# Autodesk Inventor assembly: Butterfly Drive Module
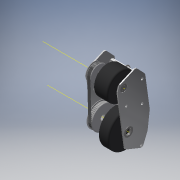
[picture p0: Inventor's stored thumbnail of the model, 180x180]
Saved by Autodesk Inventor 2019.4 (Build 234330000, 330)
## iProperties
Created: 2019-11-02
Part Number: Butterfly Drive Module
Document SubType Name: Assembly
Designer: admin
Author: admin
## Documents named in this file (12)
- C:\Users\admin\Desktop\FRC 2020 Engineering\GitHub\7738-CAD-prep\Butterfly Drive Mk2\Butterfly Module\Butterfly Drive Module.iam
- C:\Users\admin\Desktop\FRC 2020 Engineering\GitHub\7738-CAD-prep\Butterfly Drive Mk2\Butterfly Module\100mm Mecanum StandIn.ipt
- C:\Users\admin\Desktop\FRC 2020 Engineering\GitHub\7738-CAD-prep\Butterfly Drive Mk2\Butterfly Module\100mm Traction Wheel StandIn.ipt
- C:\Users\admin\Desktop\FRC 2020 Engineering\GitHub\7738-CAD-prep\Butterfly Drive Mk2\Butterfly Module\Connector.ipt
- C:\Users\admin\Desktop\FRC 2020 Engineering\GitHub\7738-CAD-prep\Butterfly Drive Mk2\Butterfly Module\F6802.ipt
- C:\Users\admin\Desktop\FRC 2020 Engineering\GitHub\7738-CAD-prep\Butterfly Drive Mk2\Butterfly Module\M6GBTeye.ipt
- C:\Users\admin\Desktop\FRC 2020 Engineering\GitHub\7738-CAD-prep\Butterfly Drive Mk2\Butterfly Module\Module Plate 1.ipt
- C:\Users\admin\Desktop\FRC 2020 Engineering\GitHub\7738-CAD-prep\Butterfly Drive Mk2\Butterfly Module\Butterfly Drive Module\Design Accelerator\Synchronous Belts Transmission1.iam
- C:\Users\admin\Desktop\FRC 2020 Engineering\GitHub\7738-CAD-prep\Butterfly Drive Mk2\Butterfly Module\Pneumatics Connector.ipt
- C:\Users\admin\Desktop\FRC 2020 Engineering\GitHub\7738-CAD-prep\Butterfly Drive Mk2\Butterfly Module\F6004.ipt
- C:\Users\admin\Desktop\FRC 2020 Engineering\GitHub\7738-CAD-prep\Butterfly Drive Mk2\Butterfly Module\Mecanum Axle.ipt
- C:\Users\admin\Desktop\FRC 2020 Engineering\GitHub\7738-CAD-prep\Butterfly Drive Mk2\Butterfly Module\Butterfly Drive Module\Design Accelerator\Key Connection1.iam
## Components (18 placed, 11 different names)
1. 100mm Mecanum StandIn:1 — Mate:2, Flush:1, Mate:19, Angle:1, Mate:43
2. 100mm Traction Wheel StandIn:1 — Mate:1, Flush:1
3. Connector:1 — Mate:5, Mate:6, Mate:10, Mate:44
4. F6802:1 — Mate:3, Mate:4, Mate:13, Mate:24, Flush:4
5. M6GBTeye:1 — Mate:9, Mate:11, Mate:33
6. Module Plate 1:1 — Mate:1, Mate:2, Mate:3, Mate:4, Mate:5, Mate:6, Mate:7, Mate:8, Mate:12, Mate:20, Mate:35, Mate:37, Mate:38, Mate:39, Mate:40, Mate:41
7. Connector:2 — Mate:7, Mate:8, Mate:9
8. M6GBTeye:2 — Mate:10, Mate:11, Flush:3
9. Synchronous Belts Transmission:1 [sub-assembly] — Mate:19, Mate:20, Mate:24, Mate:28, Mate:29, Mate:31, Angle:1
10. F6802:2 — Mate:42
11. Pneumatics Connector:1 — Mate:33, Flush:3, Mate:49
12. F6004:2 — Mate:35, Mate:37
13. Connector:3 — Mate:38, Mate:39, Mate:45, Mate:46
14. Connector:4 — Mate:40, Mate:41
15. Mecanum Axle:1 — Mate:42, Flush:4, Mate:43
16. Key Connection:1 [sub-assembly]
17. Module Plate 1:2 — Mate:44, Mate:45, Mate:46, Mate:47, Mate:48, Mate:49
18. F6004:3 — Mate:47, Mate:48
## Relationships (42: Mate 38, Flush 3, Angle 1)
- Mate:1: 100mm Traction Wheel StandIn:1 ↔ Module Plate 1:1
- Mate:2: 100mm Mecanum StandIn:1 ↔ Module Plate 1:1
- Mate:3: F6802:1 ↔ Module Plate 1:1
- Mate:4 (0.3 mm): F6802:1 ↔ Module Plate 1:1
- Mate:5: Connector:1 ↔ Module Plate 1:1
- Mate:6 (0.3 mm): Connector:1 ↔ Module Plate 1:1
- Mate:7: Module Plate 1:1 ↔ Connector:2
- Mate:8 (0.3 mm): Module Plate 1:1 ↔ Connector:2
- Mate:9: M6GBTeye:1 ↔ Connector:2
- Mate:10: Connector:1 ↔ M6GBTeye:2
- Mate:11: M6GBTeye:1 ↔ M6GBTeye:2
- Flush:1: 100mm Mecanum StandIn:1 ↔ 100mm Traction Wheel StandIn:1
- Mate:12: Module Plate 1:1
- Mate:13: F6802:1
- Mate:14
- Mate:15
- Mate:19 (3 mm): 100mm Mecanum StandIn:1 ↔ Synchronous Belts Transmission:1
- Mate:20 (3 mm): Module Plate 1:1 ↔ Synchronous Belts Transmission:1
- Mate:24: F6802:1 ↔ Synchronous Belts Transmission:1
- Mate:28: Synchronous Belts Transmission:1
- Mate:29: Synchronous Belts Transmission:1
- Mate:30
- Mate:31: Synchronous Belts Transmission:1
- Mate:32
- Mate:33: M6GBTeye:1 ↔ Pneumatics Connector:1
- Flush:3 (2 mm): M6GBTeye:2 ↔ Pneumatics Connector:1
- Mate:35: Module Plate 1:1 ↔ F6004:2
- Mate:37 (0.3 mm): Module Plate 1:1 ↔ F6004:2
- Mate:38: Module Plate 1:1 ↔ Connector:3
- Mate:39 (0.3 mm): Module Plate 1:1 ↔ Connector:3
- Mate:40: Module Plate 1:1 ↔ Connector:4
- Mate:41 (0.3 mm): Module Plate 1:1 ↔ Connector:4
- Mate:42: F6802:2 ↔ Mecanum Axle:1
- Flush:4: F6802:1 ↔ Mecanum Axle:1
- Angle:1 (0 deg): 100mm Mecanum StandIn:1 ↔ Synchronous Belts Transmission:1
- Mate:43: 100mm Mecanum StandIn:1 ↔ Mecanum Axle:1
- Mate:44: Connector:1 ↔ Module Plate 1:2
- Mate:45: Connector:3 ↔ Module Plate 1:2
- Mate:46 (0.3 mm): Connector:3 ↔ Module Plate 1:2
- Mate:47: Module Plate 1:2 ↔ F6004:3
- Mate:48 (0.3 mm): Module Plate 1:2 ↔ F6004:3
- Mate:49 (52.5 mm): Pneumatics Connector:1 ↔ Module Plate 1:2
